# Autodesk Inventor assembly: ClampedHeadbar
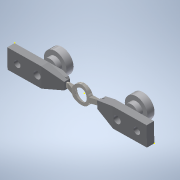
[picture p0: Inventor's stored thumbnail of the model, 180x180]
Saved by Autodesk Inventor 2022 (Build 260153000, 153)
## iProperties
Created: 2015-11-18
Part Number: ClampedHeadbar
Document SubType Name: Assembly
Designer: Vervaeke-Lab
Author: Vervaeke-Lab
## Documents named in this file (4)
- E:\Dropbox (UIO Physiology Dropbox)\Lab Data\Eivind Hennestad\Projects\AHV\Setup\Inventor Project\Assembly-ClampedHeadbar.iam
- E:\Dropbox (UIO Physiology Dropbox)\Lab Data\Eivind Hennestad\Projects\AHV\Setup\Inventor Project\Parts - HeadbarFixation\Custom-Headbar-OShape.ipt
- E:\Dropbox (UIO Physiology Dropbox)\Lab Data\Eivind Hennestad\Projects\AHV\Setup\Inventor Project\Parts - HeadbarFixation\HeadBarClamp.iam
- E:\Dropbox (UIO Physiology Dropbox)\Lab Data\Eivind Hennestad\Projects\AHV\Setup\Inventor Project\Parts - HeadbarFixation\HeadbarClampBottom.ipt
## Components (5 placed, 3 different names)
1. Custom-Headbar-OShape:1 — Mate:3, Mate:4, Mate:5, Mate:6, Angle:1, Angle:2, Mate:7, Flush:1, Mate:9, Mate:11
2. HeadBarClamp:1 [sub-assembly] — Mate:4, Mate:6, Angle:2, Mate:7, Mate:8, Flush:2
3. HeadBarClamp:2 [sub-assembly] — Mate:3, Mate:5, Angle:1, Flush:1, Mate:10, Flush:3
4. HeadbarClampBottom:1 — Mate:8, Mate:9, Flush:2
5. HeadbarClampBottom:2 — Mate:10, Mate:11, Flush:3
## Relationships (14: Mate 9, Flush 3, Angle 2)
- Mate:3: Custom-Headbar-OShape:1 ↔ HeadBarClamp:2
- Mate:4: Custom-Headbar-OShape:1 ↔ HeadBarClamp:1
- Mate:5 (-1.8 mm): Custom-Headbar-OShape:1 ↔ HeadBarClamp:2
- Mate:6 (-1.8 mm): Custom-Headbar-OShape:1 ↔ HeadBarClamp:1
- Angle:1 (0 deg): Custom-Headbar-OShape:1 ↔ HeadBarClamp:2
- Angle:2 (0 deg): Custom-Headbar-OShape:1 ↔ HeadBarClamp:1
- Mate:7: Custom-Headbar-OShape:1 ↔ HeadBarClamp:1
- Flush:1: Custom-Headbar-OShape:1 ↔ HeadBarClamp:2
- Mate:8: HeadBarClamp:1 ↔ HeadbarClampBottom:1
- Mate:9: Custom-Headbar-OShape:1 ↔ HeadbarClampBottom:1
- Flush:2 (-3.1 mm): HeadBarClamp:1 ↔ HeadbarClampBottom:1
- Mate:10: HeadBarClamp:2 ↔ HeadbarClampBottom:2
- Mate:11: Custom-Headbar-OShape:1 ↔ HeadbarClampBottom:2
- Flush:3 (-3.1 mm): HeadBarClamp:2 ↔ HeadbarClampBottom:2
